# Autodesk Inventor assembly: structure
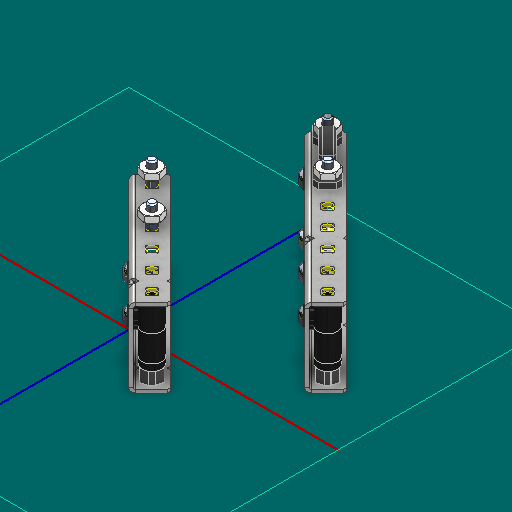
[picture p0: Inventor's stored thumbnail of the model, 512x512]
Saved by Autodesk Inventor 2025 (Build 290162000, 162)
## iProperties
Created: 2024-08-17
Part Number: structure
Document SubType Name: Assembly
Designer: averey
Author: averey
## Documents named in this file (13)
- C:\Users\avere\vex_robotics_high_stakes\hardware\cad\ATLAS\chassis\drive_pod\front_right\structure.iam
- C:\Users\avere\vex_robotics_high_stakes\hardware\cad\VEX-CAD-Inventor\Structure\C Channel\Aluminum 1x3x1\Alu C 1x3x1x6.ipt
- C:\Users\avere\vex_robotics_high_stakes\hardware\cad\_quick_assemblies\bearing_flat_w_hardware.iam
- C:\Users\avere\vex_robotics_high_stakes\hardware\cad\VEX-CAD-Inventor\Motion\Spacers\Spacer Nylon .375 OD\NSpacer .375 OD x .500.ipt
- C:\Users\avere\vex_robotics_high_stakes\hardware\cad\VEX-CAD-Inventor\Motion\Spacers\Spacer Nylon .375 OD.ipt
- C:\Users\avere\vex_robotics_high_stakes\hardware\cad\VEX-CAD-Inventor\Motion\Spacers\Spacer Nylon .375 OD\NSpacer .375 OD x .125.ipt
- C:\Users\avere\vex_robotics_high_stakes\hardware\cad\VEX-CAD-Inventor\Motion\Shaft LS\Bearing Flat Low Profile.ipt
- C:\Users\avere\vex_robotics_high_stakes\hardware\cad\VEX-CAD-Inventor\Structure\C Channel\Aluminum 1x3x1\Alu C 1x3x1x8.ipt
- C:\Users\avere\vex_robotics_high_stakes\hardware\cad\VEX-CAD-Inventor\Motion\Shaft LS\LS Pillow Bearing Block.ipt
- C:\Users\avere\vex_robotics_high_stakes\hardware\cad\VEX-CAD-Inventor\Structure\Hardware\Screw Shoulder Robosource\SScrew Shoulder Smooth .500 x .18.ipt
- C:\Users\avere\vex_robotics_high_stakes\hardware\cad\VEX-CAD-Inventor\Structure\Hardware\Screw Shoulder Robosource.ipt
- C:\Users\avere\vex_robotics_high_stakes\hardware\cad\VEX-CAD-Inventor\Structure\Hardware\Nut Nylon\Nut Nylon - White.ipt
- C:\Users\avere\vex_robotics_high_stakes\hardware\cad\VEX-CAD-Inventor\Structure\Hardware\Nut Nylon.ipt
## Components (22 placed, 9 different names)
1. Alu C 1x3x1x6:1 — Mate:1, Angle:1, Angle:2, Mate:2, Insert:1, Mate:3, Insert:5, Mate:4, Insert:6, Mate:5, Insert:16, Insert:17
2. bearing_flat_w_hardware:1 [sub-assembly] — Insert:1, Mate:3
3. NSpacer .375 OD x .500:1 — Insert:5
4. NSpacer .375 OD x .500:2
5. NSpacer .375 OD x .125:3
6. Bearing Flat Low Profile:1 — Mate:4
7. Alu C 1x3x1x8:1 — Insert:6, Mate:5, Insert:7, Mate:6, Insert:8, Mate:7, Insert:9, Mate:8, Insert:13, Mate:9, Insert:20, Insert:21
8. bearing_flat_w_hardware:2 [sub-assembly] — Insert:7, Mate:6
9. bearing_flat_w_hardware:3 [sub-assembly] — Insert:8, Mate:7
10. LS Pillow Bearing Block:1 — Insert:9, Mate:8
11. NSpacer .375 OD x .500:4
12. NSpacer .375 OD x .500:5
13. NSpacer .375 OD x .125:6
14. Bearing Flat Low Profile:2 — Insert:13, Mate:9
15. SScrew Shoulder Smooth .500 x .18:1 — Insert:17
16. Nut Nylon - White:1
17. SScrew Shoulder Smooth .500 x .18:2 — Insert:16
18. Nut Nylon - White:2
19. SScrew Shoulder Smooth .500 x .18:3 — Insert:21
20. Nut Nylon - White:3
21. SScrew Shoulder Smooth .500 x .18:4 — Insert:20
22. Nut Nylon - White:4
## Relationships (32: Insert 21, Mate 9, Angle 2)
- Mate:1 (6.35 mm): Alu C 1x3x1x6:1
- Angle:1 (0 deg): Alu C 1x3x1x6:1
- Angle:2 (45 deg): Alu C 1x3x1x6:1
- Mate:2: Alu C 1x3x1x6:1
- Insert:1: Alu C 1x3x1x6:1 ↔ bearing_flat_w_hardware:1
- Mate:3: Alu C 1x3x1x6:1 ↔ bearing_flat_w_hardware:1
- [Insert]: NSpacer .375 OD x .500:1 ↔ NSpacer .375 OD x .500:2
- [Insert]: NSpacer .375 OD x .500:2 ↔ NSpacer .375 OD x .125:3
- [Insert] (1.27 mm): NSpacer .375 OD x .125:3 ↔ Bearing Flat Low Profile:1
- Insert:5: Alu C 1x3x1x6:1 ↔ NSpacer .375 OD x .500:1
- Mate:4: Alu C 1x3x1x6:1 ↔ Bearing Flat Low Profile:1
- Insert:6 (58.7375 mm): Alu C 1x3x1x6:1 ↔ Alu C 1x3x1x8:1
- Mate:5: Alu C 1x3x1x6:1 ↔ Alu C 1x3x1x8:1
- Insert:7: Alu C 1x3x1x8:1 ↔ bearing_flat_w_hardware:2
- Mate:6: Alu C 1x3x1x8:1 ↔ bearing_flat_w_hardware:2
- Insert:8: Alu C 1x3x1x8:1 ↔ bearing_flat_w_hardware:3
- Mate:7: Alu C 1x3x1x8:1 ↔ bearing_flat_w_hardware:3
- Insert:9 (1.5875 mm): Alu C 1x3x1x8:1 ↔ LS Pillow Bearing Block:1
- Mate:8: Alu C 1x3x1x8:1 ↔ LS Pillow Bearing Block:1
- [Insert]: NSpacer .375 OD x .500:4 ↔ NSpacer .375 OD x .500:5
- [Insert]: NSpacer .375 OD x .500:5 ↔ NSpacer .375 OD x .125:6
- [Insert] (1.27 mm): NSpacer .375 OD x .125:6 ↔ Bearing Flat Low Profile:2
- Insert:13: Alu C 1x3x1x8:1 ↔ Bearing Flat Low Profile:2
- Mate:9: Alu C 1x3x1x8:1 ↔ Bearing Flat Low Profile:2
- [Insert] (6.35 mm): SScrew Shoulder Smooth .500 x .18:1 ↔ Nut Nylon - White:1
- [Insert] (6.35 mm): SScrew Shoulder Smooth .500 x .18:2 ↔ Nut Nylon - White:2
- Insert:16: Alu C 1x3x1x6:1 ↔ SScrew Shoulder Smooth .500 x .18:2
- Insert:17: Alu C 1x3x1x6:1 ↔ SScrew Shoulder Smooth .500 x .18:1
- [Insert] (6.35 mm): SScrew Shoulder Smooth .500 x .18:3 ↔ Nut Nylon - White:3
- [Insert] (6.35 mm): SScrew Shoulder Smooth .500 x .18:4 ↔ Nut Nylon - White:4
- Insert:20: Alu C 1x3x1x8:1 ↔ SScrew Shoulder Smooth .500 x .18:4
- Insert:21: Alu C 1x3x1x8:1 ↔ SScrew Shoulder Smooth .500 x .18:3
## Named parameters: d57_d39_d36 = 0 mm, d58_d51 = 0 mm, d59_d56 = 1.27 mm, d19_d57_d39_d36 = 0 mm, d20_d58_d51 = 0 mm, d21_d59_d56 = 1.27 mm, d48_d44 = 6.35 mm, d25_d48_d44 = 6.35 mm, d28_d48_d44 = 6.35 mm, d29_d48_d44 = 6.35 mm
